# Autodesk Inventor assembly: 大粗轴四方轴套反
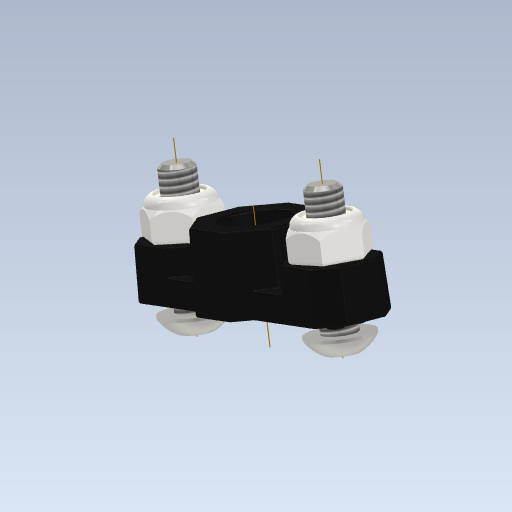
[picture p0: Inventor's stored thumbnail of the model, 512x512]
Saved by Autodesk Inventor 2020 (Build 240168000, 168)
## iProperties
Created: 2019-05-29
Part Number: 大粗轴四方轴套反
Document SubType Name: Assembly
Designer: aresp
Author: aresp
## Documents named in this file (3)
- D:\vault\ncrCadLib\轴相关\粗轴配套\大粗轴四方轴套反.iam
- D:\vault\ncrCadLib\轴相关\粗轴配套\零件\大粗轴四方轴套.ipt
- D:\vault\ncrCadLib\轴相关\粗轴配套\零件\四号螺丝+防滑.iam
## Components (3 placed, 2 different names)
1. 大粗轴四方轴套:1 — 配合:2, 配合:6, 螺丝粘合轴承片正, 螺丝粘合轴承片反
2. 四号螺丝+防滑:1 [sub-assembly] — 配合:2, 表面齐平:1, 螺丝粘合轴承片正, 螺丝粘合轴承片反
3. 四号螺丝+防滑:2 [sub-assembly] — 配合:6, 表面齐平:1
## Relationships (5: Mate 4, Flush 1)
- 配合:2 [Mate]: 大粗轴四方轴套:1 ↔ 四号螺丝+防滑:1
- 配合:6 [Mate]: 大粗轴四方轴套:1 ↔ 四号螺丝+防滑:2
- 表面齐平:1 [Flush]: 四号螺丝+防滑:1 ↔ 四号螺丝+防滑:2
- 螺丝粘合轴承片正 [Mate]: 大粗轴四方轴套:1 ↔ 四号螺丝+防滑:1
- 螺丝粘合轴承片反 [Mate]: 大粗轴四方轴套:1 ↔ 四号螺丝+防滑:1
